# Autodesk Inventor assembly: pihti-for-simulation-flat
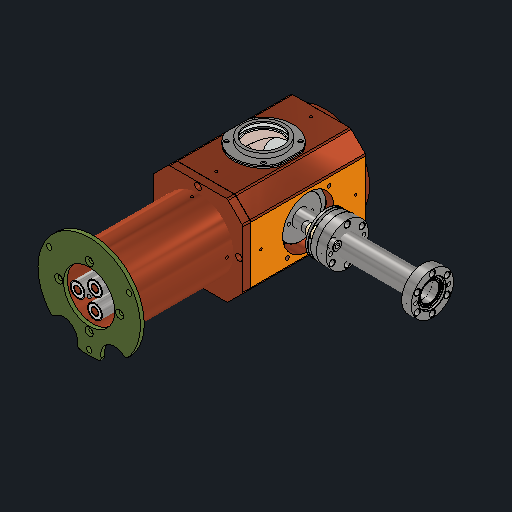
[picture p0: Inventor's stored thumbnail of the model, 512x512]
Saved by Autodesk Inventor 2027.1 (Build 311270010, 270A)
## iProperties
Created: 2026-10-01
Part Number: pihti-for-simulation-flat
Document SubType Name: Assembly
Designer: queezz
Author: queezz
## Documents named in this file (51)
- C:\Users\queezz\Dropbox\Drawings\pihti-cad\Plasma Vessel\pihti-for-simulation-flat.iam
- C:\Users\queezz\Dropbox\Drawings\pihti-cad\Plasma Vessel\Plasma-Flange-2024\cathode-box.ipt
- C:\Users\queezz\Dropbox\Drawings\pihti-cad\Plasma Vessel\Plasma-Flange-2024\cathode-box-mounting-plate.ipt
- C:\Users\queezz\Dropbox\Drawings\pihti-cad\Plasma Vessel\Cathode-Anode-Flange\copper-feed\HighCurrentFeed_Ceramic-insulator.ipt
- C:\Users\queezz\Dropbox\Drawings\pihti-cad\Plasma Vessel\Cathode-Anode-Flange\copper-feed\HighCurrentFeed_connecting-bushing.ipt
- C:\Users\queezz\Dropbox\Drawings\pihti-cad\Plasma Vessel\Cathode-Anode-Flange\copper-feed\HighCurrentFeed_welded-plate-top.ipt
- C:\Users\queezz\Dropbox\Drawings\pihti-cad\Plasma Vessel\Cathode-Anode-Flange\copper-feed\HighCurrentFeedRod.ipt
- C:\Users\queezz\Dropbox\Drawings\pihti-cad\ContentCenter\Fastners\m5-nut.ipt
- C:\Users\queezz\Dropbox\Drawings\pihti-cad\Plasma Vessel\Cathode-Anode-Flange\ring-pre-anode.ipt
- C:\Users\queezz\Dropbox\Drawings\pihti-cad\Plasma Vessel\Cathode-Anode-Flange\cathode-screen-v0.ipt
- C:\Users\queezz\Dropbox\Drawings\pihti-cad\Plasma Vessel\Cathode-Anode-Flange\electrode-skirt-pipe.ipt
- C:\Users\queezz\Dropbox\Drawings\pihti-cad\Plasma Vessel\Cathode-Anode-Flange\electrode-aligning-disk.ipt
- C:\Users\queezz\Dropbox\Drawings\pihti-cad\Plasma Vessel\Cathode-Anode-Flange\m3-pin-for-ring-anode.ipt
- C:\Users\queezz\Dropbox\Drawings\pihti-cad\ContentCenter\Fastners\M3-nut.ipt
- C:\Users\queezz\Dropbox\Drawings\pihti-cad\Plasma Vessel\Cathode-Anode-Flange\m3-pin-for-cathode-skirt.ipt
- C:\Users\queezz\Dropbox\Drawings\pihti-cad\Plasma Vessel\Cathode-Anode-Flange\anode-holding-nut.ipt
- C:\Users\queezz\Dropbox\Drawings\pihti-cad\Plasma Vessel\Cathode-Anode-Flange\electrode-skirt-short.ipt
- C:\Users\queezz\Dropbox\Drawings\pihti-cad\Plasma Vessel\Cathode-Anode-Flange\Cathode-tungsten-wire-v3-filament-solid.ipt
- C:\Users\queezz\Dropbox\Drawings\pihti-cad\Plasma Vessel\Plasma-Box\plasma_box.ipt
- C:\Users\queezz\Dropbox\Drawings\pihti-cad\Plasma Vessel\Plasma-Box\probe-gate-spacer.ipt
- C:\Users\queezz\Dropbox\Drawings\pihti-cad\Plasma Vessel\Plasma-Box\plasma-box-slit-to-cathode.ipt
- C:\Users\queezz\Dropbox\Drawings\pihti-cad\Plasma Vessel\Plasma-Box\probe-gate-spacer\probe-gate-spacer-quartz-holder.ipt
- C:\Users\queezz\Dropbox\Drawings\pihti-cad\Plasma Vessel\Plasma-Box\quartz-disk-window.ipt
- C:\Users\queezz\Dropbox\Drawings\pihti-cad\Plasma Vessel\Plasma-Box\quartz-disk-window-holder.ipt
- C:\Users\queezz\Dropbox\Drawings\pihti-cad\Plasma Vessel\Plasma-Box\probe-gate-spacer\probe-gate-spacer-40mm-mesh-holder.ipt
- C:\Users\queezz\Dropbox\Drawings\pihti-cad\Plasma Vessel\Plasma-Box\plasma-box-spacer-6mm.ipt
- C:\Users\queezz\Dropbox\Drawings\pihti-cad\Plasma Vessel\Plasma-Box\plasma-box-mica.ipt
- C:\Users\queezz\Dropbox\Drawings\pihti-cad\Plasma Vessel\Boron-Target\boron-dish.ipt
- C:\Users\queezz\Dropbox\Drawings\pihti-cad\Plasma Vessel\Boron-Target\skirt-cylinder.ipt
- C:\Users\queezz\Dropbox\Drawings\pihti-cad\Plasma Vessel\Boron-Target\skirt-base.ipt
- C:\Users\queezz\Dropbox\Drawings\pihti-cad\ContentCenter\Ceramics\ceramic_bushing_M3-v1.ipt
- C:\Users\queezz\Dropbox\Drawings\pihti-cad\ContentCenter\Ceramics\ceramic_washer_M4_v1.ipt
- C:\Users\queezz\Dropbox\Drawings\pihti-cad\Plasma Vessel\Boron-Target\m3-pin-boron.ipt
- C:\Users\queezz\Dropbox\Drawings\pihti-cad\Plasma Vessel\Boron-Target\skirt-lid-for-grooved-targetr.ipt
- C:\Users\queezz\Dropbox\Drawings\pihti-cad\Plasma Vessel\Boron-Target\mesh.ipt
- C:\Users\queezz\Dropbox\Drawings\pihti-cad\Plasma Vessel\Boron-Target\boron-under-mesh-plate.ipt
- C:\Users\queezz\Dropbox\Drawings\pihti-cad\Plasma Vessel\Boron-Target\boron-window.ipt
- C:\Users\queezz\Dropbox\Drawings\pihti-cad\Plasma Vessel\Plasma-Box\anode_holder.ipt
- C:\Users\queezz\Dropbox\Drawings\pihti-cad\Plasma Vessel\Plasma-Box\anode-disk.ipt
- C:\Users\queezz\Dropbox\Drawings\pihti-cad\Plasma Vessel\Plasma-Box\anode-m4-threaded-rod.ipt
- C:\Users\queezz\Dropbox\Drawings\pihti-cad\ContentCenter\Ceramics\ceramic_bushing_M4.ipt
- C:\Users\queezz\Dropbox\Drawings\pihti-cad\ContentCenter\Fastners\M4-nut.ipt
- C:\Users\queezz\Dropbox\Drawings\pihti-cad\Plasma Vessel\Plasma-Box\probe-side-large-mesh.ipt
- C:\Users\queezz\Dropbox\Drawings\pihti-cad\Plasma Vessel\probe-port-mesh.ipt
- C:\Users\queezz\Dropbox\Drawings\pihti-cad\Plasma Vessel\pihti-simulation-ceramic-sleeve-10x6x110.ipt
- C:\Users\queezz\Dropbox\Drawings\pihti-cad\Plasma Vessel\Cathode-Anode-Flange\preanode-screen.ipt
- C:\Users\queezz\Dropbox\Drawings\pihti-cad\Plasma Vessel\Cathode-Anode-Flange\ingnition-help.ipt
- C:\Users\queezz\Dropbox\Drawings\pihti-cad\Plasma Vessel\ignition-alumina-tube-lower.ipt
- C:\Users\queezz\Dropbox\Drawings\pihti-cad\Plasma Vessel\ignition-alumina-tube-upper.ipt
- C:\Users\queezz\Dropbox\Drawings\pihti-cad\BoronProbe\BoronHead.iam
- C:\Users\queezz\Dropbox\Drawings\pihti-cad\staging\sample-holder-base-hayashi.ipt
## Components (64 placed, 49 different names)
1. cathode-box:2
2. cathode-box-mounting-plate:3
3. HighCurrentFeed_Ceramic-insulator:27
4. HighCurrentFeed_connecting-bushing:28
5. HighCurrentFeed_welded-plate-top:29
6. HighCurrentFeedRod:30 — Mate:1
7. HighCurrentFeed_Ceramic-insulator:31
8. HighCurrentFeed_connecting-bushing:32
9. HighCurrentFeed_welded-plate-top:33
10. HighCurrentFeedRod:34
11. HighCurrentFeed_Ceramic-insulator:35
12. HighCurrentFeed_connecting-bushing:36
13. HighCurrentFeed_welded-plate-top:37
14. HighCurrentFeedRod:38
15. m5-nut:40
16. m5-nut:41
17. m5-nut:42
18. ring-pre-anode:79
19. cathode-screen-v0:80
20. electrode-skirt-pipe:81
21. electrode-skirt-pipe:82 — Mate:4
22. electrode-skirt-pipe:83
23. electrode-aligning-disk:85 — Mate:3
24. m3-pin-for-ring-anode:86 — Mate:2, Mate:5
25. m3-pin-for-cathode-skirt:89
26. anode-holding-nut:95 — Mate:1, Mate:2, Mate:6
27. electrode-skirt-short:102
28. electrode-skirt-short:103
29. Cathode-tungsten-wire-v3-filament-solid:104
30. plasma_box:105 — Mate:12
31. plasma-box-slit-to-cathode:117
32. probe-gate-spacer-quartz-holder:120
33. quartz-disk-window:121
34. quartz-disk-window-holder:122
35. plasma-box-spacer-6mm:129
36. plasma-box-mica:137
37. anode_holder:160
38. anode-disk:161
39. anode-m4-threaded-rod:162
40. ceramic_bushing_M4:164
41. M4-nut:165
42. preanode-screen:1 — Mate:3, Mate:4, preanode-screen XZ through assembly Z
43. ingnition-help:1 — Mate:5, Mate:6, ingnition-help XZ through assembly Z
44. Ignition-alumina-lower:1
45. Ignition-alumina-upper:1
46. BoronHead:1 [sub-assembly] — Mate:9, Mate:10, Mate:11, Mate:12
47. sample-holder-base-hayashi:1 — Mate:9, Mate:10, Mate:11, Mate:13
48. Cathode-feed-ceramic-sleeve:3
49. Cathode-feed-ceramic-sleeve:2
50. Cathode-feed-ceramic-sleeve:1
51. boron-dish:138
52. skirt-cylinder:139 — Mate:13
53. skirt-base:140
54. ceramic_bushing_M3-v1:141
55. ceramic_washer_M4_v1:142
56. m3-pin-boron:143
57. M3-nut:144
58. skirt-lid-for-grooved-targetr:146
59. mesh:147
60. boron-under-mesh-plate:148
61. boron-window:149
62. probe-gate-spacer-40mm-mesh-holder:123
63. probe-side-large-mesh:175
64. probe-port-mesh:180
## Relationships (13: Mate 13)
- Mate:1: HighCurrentFeedRod:30 ↔ anode-holding-nut:95
- Mate:2: m3-pin-for-ring-anode:86 ↔ anode-holding-nut:95
- Mate:3: electrode-aligning-disk:85 ↔ preanode-screen:1
- Mate:4: electrode-skirt-pipe:82 ↔ preanode-screen:1
- Mate:5: m3-pin-for-ring-anode:86 ↔ ingnition-help:1
- Mate:6 (15 mm): anode-holding-nut:95 ↔ ingnition-help:1
- preanode-screen XZ through assembly Z [Mate]: preanode-screen:1
- ingnition-help XZ through assembly Z [Mate]: ingnition-help:1
- Mate:9: BoronHead:1 ↔ sample-holder-base-hayashi:1
- Mate:10: BoronHead:1 ↔ sample-holder-base-hayashi:1
- Mate:11: BoronHead:1 ↔ sample-holder-base-hayashi:1
- Mate:12: plasma_box:105 ↔ BoronHead:1
- Mate:13: sample-holder-base-hayashi:1 ↔ skirt-cylinder:139
